# Autodesk Inventor assembly: Firgelli L16 50mm Assembly
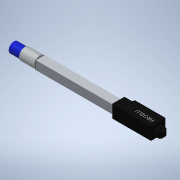
[picture p0: Inventor's stored thumbnail of the model, 180x180]
Saved by Autodesk Inventor 2020 (Build 240168000, 168)
## iProperties
Created: 2017-11-30
Part Number: Firgelli L16 50mm Assembly
Document SubType Name: Assembly
Designer: stedrock
Sending System: SolidWorks 2014-2014161
MC: AMD64
MC_MODEL: Intel64 Family 6 Model 23 Stepping 10, GenuineIntel
OS: Windows_NT
FRU: Parasolid Version 25.1, build 231,  3-13-2014
FORMAT: text
GUISE: transmit
KEY: Firgelli L16 50mm Assembly
FILE: Firgelli L16 50mm Assembly.x_t
DATE: Thu Jul 10 09:01:34 2014
Author: stedrock
## Documents named in this file (3)
- C:\Users\jous\Desktop\boat\actuator\Firgelli L16 50mm Assembly.iam
- C:\Users\jous\Desktop\boat\actuator\Firgelli L16 50mm body(50).ipt
- C:\Users\jous\Desktop\boat\actuator\Firgelli L16 50mm as(Short).ipt
## Components (2 placed, 2 different names)
1. Firgelli L16 50mm body(50) — Rotational:3
2. Firgelli L16 50mm as(Short) — Rotational:3
## Relationships (1: RevoluteJoint 1)
- Rotational:3 [RevoluteJoint] (51.196 mm): Firgelli L16 50mm body(50) ↔ Firgelli L16 50mm as(Short)
